# Autodesk Inventor assembly: Motor_Valve_Assembly
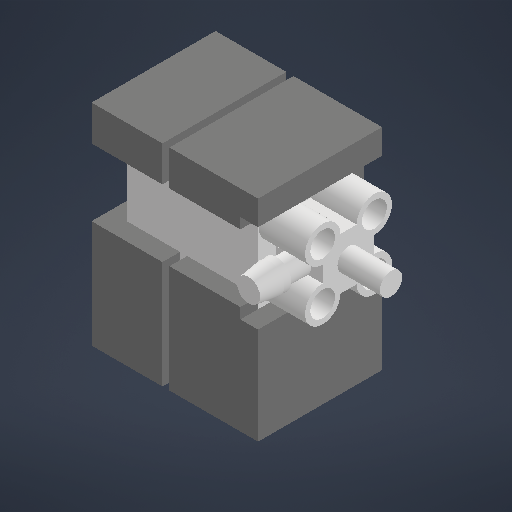
[picture p0: Inventor's stored thumbnail of the model, 512x512]
Saved by Autodesk Inventor 2026.2 (Build 302298000, 298)
## iProperties
Created: 2026-02-03
Part Number: Motor_Valve_Assembly
Document SubType Name: Assembly
Designer: vckot
Author: vckot
## Documents named in this file (4)
- C:\Users\vckot\OneDrive\Documents\Vaibhav\capstone\CAD_files\Motor_Valve\Motor_Valve_Assembly.iam
- C:\Users\vckot\OneDrive\Documents\Vaibhav\capstone\CAD_files\Motor_Valve\Adafruit_1528-4663-ND.ipt
- C:\Users\vckot\OneDrive\Documents\Vaibhav\capstone\CAD_files\Motor_Valve\Adafruit_1528_4663-ND_House_01.ipt
- C:\Users\vckot\OneDrive\Documents\Vaibhav\capstone\CAD_files\Motor_Valve\Adafruit_1528_4663-ND_House_02.ipt
## Components (3 placed, 3 different names)
1. Adafruit_1528-4663-ND:1 — Mate:1, Mate:2, Mate:3, Mate:4, Mate:5, Mate:6
2. Adafruit_1528_4663-ND_House_01:1 — Mate:1, Mate:2, Mate:3
3. Adafruit_1528_4663-ND_House_02:1 — Mate:4, Mate:5, Mate:6
## Relationships (6: Mate 6)
- Mate:1: Adafruit_1528-4663-ND:1 ↔ Adafruit_1528_4663-ND_House_01:1
- Mate:2: Adafruit_1528-4663-ND:1 ↔ Adafruit_1528_4663-ND_House_01:1
- Mate:3: Adafruit_1528-4663-ND:1 ↔ Adafruit_1528_4663-ND_House_01:1
- Mate:4: Adafruit_1528-4663-ND:1 ↔ Adafruit_1528_4663-ND_House_02:1
- Mate:5: Adafruit_1528-4663-ND:1 ↔ Adafruit_1528_4663-ND_House_02:1
- Mate:6: Adafruit_1528-4663-ND:1 ↔ Adafruit_1528_4663-ND_House_02:1
